# Autodesk Inventor assembly: Assembly_Cube_Eyeball_v3
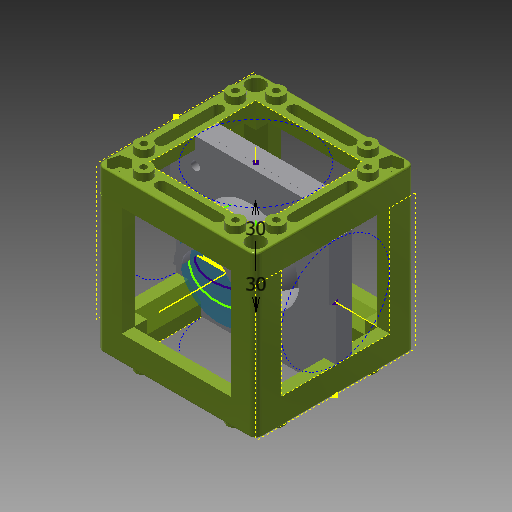
[picture p0: Inventor's stored thumbnail of the model, 512x512]
Saved by Autodesk Inventor 2019 (Build 230136000, 136)
## iProperties
Created: 2020-02-04
Part Number: Assembly_Cube_Eyeball_v3
Document SubType Name: Assembly
Designer: marsikovabarbora
Author: marsikovabarbora
## Documents named in this file (5)
- C:\Users\marsikovabarbora\Dropbox\UC2\02_CAD\INVENTOR\uc2_v3\Assembly_Cube_Eyeball_v3.iam
- C:\Users\marsikovabarbora\Dropbox\UC2\02_CAD\INVENTOR\uc2_v3\20_Cube_Insert_Eye_v3.ipt
- C:\Users\marsikovabarbora\Dropbox\UC2\02_CAD\INVENTOR\uc2_v3\20_Cube_Insert_Eye_Lens_v3.ipt
- C:\Users\marsikovabarbora\Dropbox\UC2\02_CAD\INVENTOR\uc2_v3\00_Lens_d21,5.ipt
- C:\Users\marsikovabarbora\Dropbox\UC2\02_CAD\INVENTOR\uc2_v3\Assembly_Cube_empty_IM_v3.iam
## Components (4 placed, 4 different names)
1. 20_Cube_Insert_Eye_v3:1 — Mate:1, Angle:1, Mate:2, Mate:3, Mate:4, Fluchtend:3, Fluchtend:4, Mate:5
2. 20_Cube_Insert_Eye_Lens_v3:1 — Mate:1, Angle:1, Mate:2, Flush:2
3. Assembly_Cube_empty_IM_v3:1 [sub-assembly] — Fluchtend:3, Fluchtend:4, Mate:5
4. 00_Lens_d21,5:1 — Flush:2
## Relationships (9: Mate 5, Flush 3, Angle 1)
- Mate:1: 20_Cube_Insert_Eye_v3:1 ↔ 20_Cube_Insert_Eye_Lens_v3:1
- Angle:1 (0 deg): 20_Cube_Insert_Eye_v3:1 ↔ 20_Cube_Insert_Eye_Lens_v3:1
- Mate:2: 20_Cube_Insert_Eye_v3:1 ↔ 20_Cube_Insert_Eye_Lens_v3:1
- Mate:3: 20_Cube_Insert_Eye_v3:1
- Mate:4: 20_Cube_Insert_Eye_v3:1
- Flush:2: 20_Cube_Insert_Eye_Lens_v3:1 ↔ 00_Lens_d21,5:1
- Fluchtend:3 [Flush]: 20_Cube_Insert_Eye_v3:1 ↔ Assembly_Cube_empty_IM_v3:1
- Fluchtend:4 [Flush]: 20_Cube_Insert_Eye_v3:1 ↔ Assembly_Cube_empty_IM_v3:1
- Mate:5: 20_Cube_Insert_Eye_v3:1 ↔ Assembly_Cube_empty_IM_v3:1
